# Autodesk Inventor assembly: 플라이휠+샤프트홀더
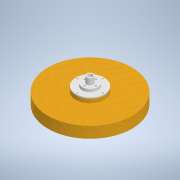
[picture p0: Inventor's stored thumbnail of the model, 180x180]
Saved by Autodesk Inventor 2020 (Build 240168000, 168)
## iProperties
Created: 2020-05-01
Part Number: 플라이휠+샤프트홀더
Document SubType Name: Assembly
Designer: introbot
Author: introbot
## Documents named in this file (4)
- C:\Users\introbot\Desktop\플라이휠+샤프트홀더2\플라이휠+샤프트홀더.iam
- C:\Users\introbot\Desktop\도면\Wheel 2.ipt
- C:\Users\introbot\Desktop\플라이휠+샤프트홀더2\판.ipt
- C:\Users\introbot\Desktop\플라이휠+샤프트홀더2\STHRB8.iam
## Components (3 placed, 3 different names)
1. Wheel 2:1 — Mate:7, Mate:8
2. 판:1 — Mate:4, Mate:5, Mate:6, Mate:7, Mate:8
3. STHRB8:1 [sub-assembly] — Mate:4, Mate:5, Mate:6
## Relationships (5: Mate 5)
- Mate:4: 판:1 ↔ STHRB8:1
- Mate:5: 판:1 ↔ STHRB8:1
- Mate:6: 판:1 ↔ STHRB8:1
- Mate:7: Wheel 2:1 ↔ 판:1
- Mate:8: Wheel 2:1 ↔ 판:1
